# Autodesk Inventor assembly: SFU1204
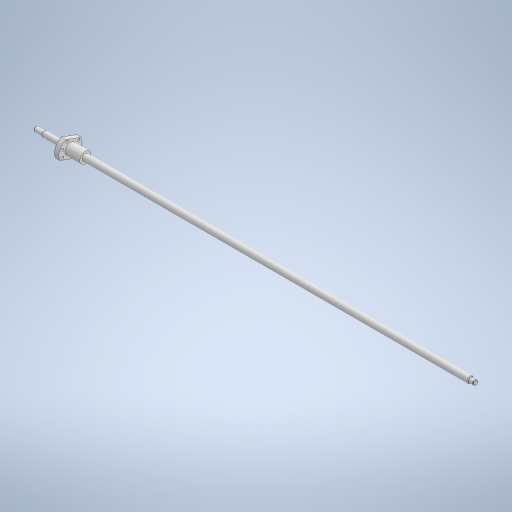
[picture p0: Inventor's stored thumbnail of the model, 512x512]
Saved by Autodesk Inventor 2023 (Build 270158000, 158)
## iProperties
Created: 2022-04-29
Part Number: SFU1204
Document SubType Name: Assembly
Designer: plebbb
Author: plebbb
## Documents named in this file (3)
- D:\Users\plebbb\Desktop\CNC_Project\SFU1204.iam
- D:\Users\plebbb\Desktop\CNC_Project\SFU1204-800.ipt
- D:\Users\plebbb\Desktop\CNC_Project\SFU1204-Housing.ipt
## Components (2 placed, 2 different names)
1. SFU1204-800:1 — Mate:1, Mate:2
2. SFU1204-Housing:1 — Mate:1, Mate:2
## Relationships (2: Mate 2)
- Mate:1: SFU1204-800:1 ↔ SFU1204-Housing:1
- Mate:2: SFU1204-800:1 ↔ SFU1204-Housing:1
